# Autodesk Inventor assembly: SUBBallValve
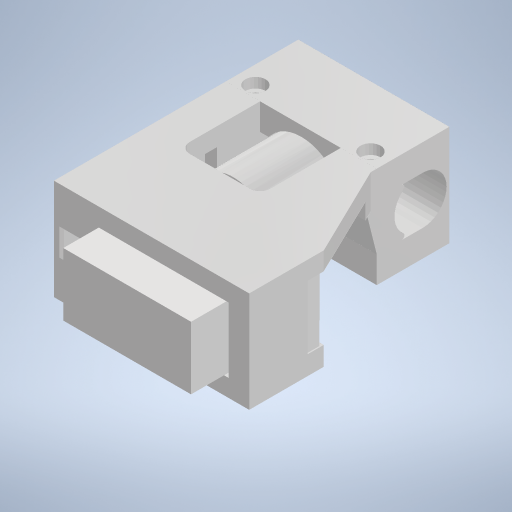
[picture p0: Inventor's stored thumbnail of the model, 512x512]
Saved by Autodesk Inventor 2024 (Build 280153000, 153)
## iProperties
Created: 2025-02-07
Part Number: SUBBallValve
Document SubType Name: Assembly
Designer: Tommy Rohmann
Author: Tommy Rohmann
## Documents named in this file (5)
- C:\Users\Tommy Rohmann\OneDrive\Projects\Microgravity-Press-Washing-Machine\System Design and Documentation\Inventor Design Project\Actuated Ball Valves\SUBBallValve.iam
- C:\Users\Tommy Rohmann\Downloads\BallValveMount.ipt
- C:\Users\Tommy Rohmann\Downloads\ServoAdapter.ipt
- C:\Users\Tommy Rohmann\Downloads\ServoMount.ipt
- C:\Users\Tommy Rohmann\OneDrive\Projects\Microgravity-Press-Washing-Machine\System Design and Documentation\Inventor Design Project\Actuated Ball Valves\ServoSimplified.ipt
## Components (4 placed, 4 different names)
1. BallValveMount:1 — Mate:4, Flush:1, Mate:5, Mate:6, Mate:7
2. ServoAdapter:1 — Mate:6, Mate:7
3. ServoMount:1 — Mate:1, Mate:2, Mate:3, Mate:4, Flush:1, Mate:5
4. ServoSimplified:1 — Mate:1, Mate:2, Mate:3
## Relationships (8: Mate 7, Flush 1)
- Mate:1: ServoMount:1 ↔ ServoSimplified:1
- Mate:2: ServoMount:1 ↔ ServoSimplified:1
- Mate:3: ServoMount:1 ↔ ServoSimplified:1
- Mate:4: BallValveMount:1 ↔ ServoMount:1
- Flush:1: BallValveMount:1 ↔ ServoMount:1
- Mate:5: BallValveMount:1 ↔ ServoMount:1
- Mate:6: BallValveMount:1 ↔ ServoAdapter:1
- Mate:7: BallValveMount:1 ↔ ServoAdapter:1
